# Autodesk Inventor assembly: Assembly12
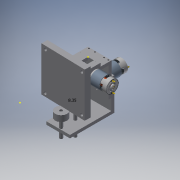
[picture p0: Inventor's stored thumbnail of the model, 180x180]
Saved by Autodesk Inventor 2019.4 (Build 234330000, 330)
## iProperties
Created: 2020-03-04
Part Number: Assembly12
Document SubType Name: Assembly
Designer: Niran
Author: Niran
## Documents named in this file (11)
- C:\Users\Niran\Desktop\sketch_jan26a\Canon parts\Assembly12.iam
- C:\Users\Niran\Desktop\sketch_jan26a\Canon parts\Part111.ipt
- C:\Users\Niran\Desktop\sketch_jan26a\Canon parts\VIRTUAL IMPLEMENTATION\rod2.ipt
- C:\Users\Niran\Desktop\sketch_jan26a\Canon parts\VIRTUAL IMPLEMENTATION\rod4.ipt
- C:\Users\Niran\Desktop\sketch_jan26a\Canon parts\VIRTUAL IMPLEMENTATION\gear_z18_m1.ipt
- C:\Users\Niran\Desktop\sketch_jan26a\Canon parts\VIRTUAL IMPLEMENTATION\wheel.ipt
- C:\Users\Niran\Desktop\sketch_jan26a\Canon parts\VIRTUAL IMPLEMENTATION\Rack.ipt
- C:\Users\Niran\Desktop\sketch_jan26a\Canon parts\carromboard15cm.ipt
- C:\Users\Niran\Desktop\sketch_jan26a\Canon parts\Part40.ipt
- C:\Users\Niran\Desktop\sketch_jan26a\Canon parts\striking.iam
- C:\Users\Niran\Desktop\sketch_jan26a\Canon parts\DC Motor.ipt
## Components (11 placed, 10 different names)
1. Part111:1 — Rigid:2, Rigid:3, Rigid:4
2. rod2:1 — Rigid:3, Rotational:2
3. rod2:2 — Rotational:1, Rigid:2
4. rod4:1 — Rigid:1, Rotational:1
5. gear_z18_m1:1 — Rigid:1, Rotational:3
6. wheel:1 — Rotational:2
7. Rack:1 — Rotational:3, Rotational:4
8. carromboard15cm:1 — Rotational:4
9. Part40:1 — Rigid:4, Rotational:5, Rotational:6
10. striking:1 [sub-assembly] — Rotational:5
11. DC Motor:1 — Rotational:6
## Relationships (10: RevoluteJoint 6, WeldJoint 4)
- Rigid:1 [WeldJoint]: rod4:1 ↔ gear_z18_m1:1
- Rotational:1 [RevoluteJoint]: rod2:2 ↔ rod4:1
- Rigid:2 [WeldJoint] (-50 mm): Part111:1 ↔ rod2:2
- Rigid:3 [WeldJoint] (-30 mm): Part111:1 ↔ rod2:1
- Rotational:2 [RevoluteJoint] (5 mm): rod2:1 ↔ wheel:1
- Rotational:3 [RevoluteJoint]: gear_z18_m1:1 ↔ Rack:1
- Rotational:4 [RevoluteJoint]: Rack:1 ↔ carromboard15cm:1
- Rigid:4 [WeldJoint]: Part111:1 ↔ Part40:1
- Rotational:5 [RevoluteJoint]: Part40:1 ↔ striking:1
- Rotational:6 [RevoluteJoint] (11 mm): Part40:1 ↔ DC Motor:1
